# Autodesk Inventor assembly: KS-15_all_cornering+air
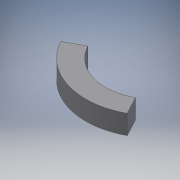
[picture p0: Inventor's stored thumbnail of the model, 180x180]
Saved by Autodesk Inventor 2018.2 (Build 222227000, 227)
## iProperties
Created: 2018-05-19
Part Number: KS-15_all_cornering+air
Material: 一般
Document SubType Name: Assembly
Designer: ku_sk
Author: ku_sk
## Documents named in this file (3)
- D:\ku_sk\ドキュメント\Inventor\Aero\KS-15\全体アッセンブリ解析用モデル\KS-15_all_cornering+air.iam
- D:\ku_sk\ドキュメント\Inventor\Aero\KS-15\全体アッセンブリ解析用モデル\KS-15_all_cornering.iam
- D:\ku_sk\ドキュメント\Inventor\Aero\KS-15\全体アッセンブリ解析用モデル\air\air_skidpad.ipt
## Components (2 placed, 2 different names)
1. air_skidpad:1 — メイト:2, フラッシュ:4, 角度:1
2. KS-15_all_cornering:1 [sub-assembly] — メイト:1, メイト:2, フラッシュ:4, 角度:1
## Relationships (4: Mate 2, Flush 1, Angle 1)
- メイト:1 [Mate]: KS-15_all_cornering:1
- メイト:2 [Mate]: air_skidpad:1 ↔ KS-15_all_cornering:1
- フラッシュ:4 [Flush] (-30 mm): air_skidpad:1 ↔ KS-15_all_cornering:1
- 角度:1 [Angle] (-2.2 deg): air_skidpad:1 ↔ KS-15_all_cornering:1
